# Autodesk Inventor assembly: nc_nhk15
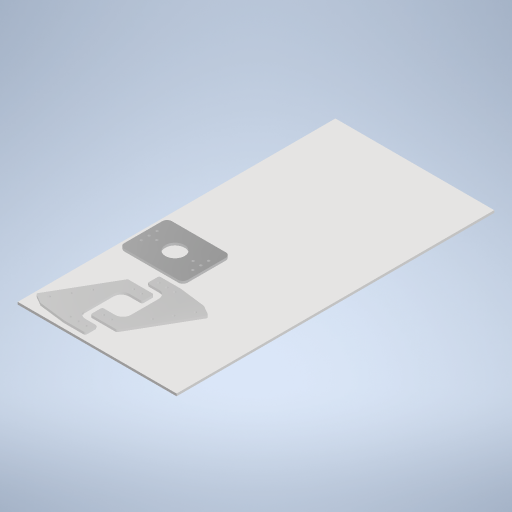
[picture p0: Inventor's stored thumbnail of the model, 512x512]
Saved by Autodesk Inventor 2023 (Build 270158000, 158)
## iProperties
Created: 2022-04-24
Part Number: nc_nhk15
Document SubType Name: Assembly
Designer: yuta
Author: yuta
## Documents named in this file (4)
- C:\Users\yuta\Documents\NHK\nc_nhk15.iam
- C:\Users\yuta\Documents\NHK\旧\NC.port.ipt
- C:\Users\yuta\Desktop\オムニホイール\ホイールユニット_側板1.ipt
- C:\Users\yuta\Documents\NHK\射出_エンコーダー固定.ipt
## Components (4 placed, 3 different names)
1. NC.port:1 — メイト:1, メイト:2, フラッシュ:1, メイト:3, メイト:6, フラッシュ:2
2. ホイールユニット_側板1:1 — メイト:1, フラッシュ:1, メイト:3, メイト:4, メイト:5
3. ホイールユニット_側板1:2 — メイト:2, メイト:4, メイト:5, メイト:7
4. 射出_エンコーダー固定:1 — メイト:6, フラッシュ:2, メイト:7
## Relationships (9: Mate 7, Flush 2)
- メイト:1 [Mate]: NC.port:1 ↔ ホイールユニット_側板1:1
- メイト:2 [Mate]: NC.port:1 ↔ ホイールユニット_側板1:2
- フラッシュ:1 [Flush] (6 mm): NC.port:1 ↔ ホイールユニット_側板1:1
- メイト:3 [Mate] (-8 mm): NC.port:1 ↔ ホイールユニット_側板1:1
- メイト:4 [Mate] (8 mm): ホイールユニット_側板1:1 ↔ ホイールユニット_側板1:2
- メイト:5 [Mate] (8 mm): ホイールユニット_側板1:1 ↔ ホイールユニット_側板1:2
- メイト:6 [Mate]: NC.port:1 ↔ 射出_エンコーダー固定:1
- フラッシュ:2 [Flush] (6 mm): NC.port:1 ↔ 射出_エンコーダー固定:1
- メイト:7 [Mate] (8 mm): ホイールユニット_側板1:2 ↔ 射出_エンコーダー固定:1
